# Autodesk Inventor assembly: Assembly5
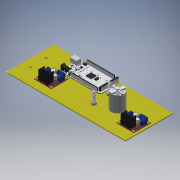
[picture p0: Inventor's stored thumbnail of the model, 180x180]
Saved by Autodesk Inventor 2019 (Build 230136000, 136)
## iProperties
Created: 2020-02-13
Part Number: Assembly5
Document SubType Name: Assembly
Designer: Dell
Author: Dell
## Documents named in this file (9)
- C:\Users\Dell\Documents\Assembly5.iam
- control.iam
- C:\Users\Dell\Documents\3dmodelling2.ipt
- C:\Users\Dell\Documents\bolt.ipt
- C:\Users\Dell\Documents\3dmodelling3.ipt
- C:\Users\Dell\Documents\nut2.ipt
- C:\Users\Dell\Documents\motordc2.ipt
- C:\Users\Dell\Documents\motordriver2.ipt
- C:\Users\Dell\Documents\arduinomega3.ipt
## Components (10 placed, 7 different names)
1. 3dmodelling2:1 — Rotational:1, Rotational:2, Rotational:3, Rotational:5, Mate:1, Mate:3
2. bolt:1 — Rotational:1
3. bolt:2 — Rotational:2, Rotational:4, Rotational:5, Rigid:1
4. 3dmodelling3:1 — Rotational:3, Rotational:4, Rotational:6, Rotational:7, Mate:2
5. nut2:1 — Rotational:6
6. nut2:2 — Rigid:1
7. motordc2:1 — Rotational:7
8. motordriver2:1 — Mate:2
9. motordriver2:2 — Mate:1
10. arduinomega3:1 — Mate:3
## Relationships (11: RevoluteJoint 7, Mate 3, WeldJoint 1)
- Rotational:1 [RevoluteJoint]: 3dmodelling2:1 ↔ bolt:1
- Rotational:2 [RevoluteJoint]: 3dmodelling2:1 ↔ bolt:2
- Rotational:3 [RevoluteJoint]: 3dmodelling2:1 ↔ 3dmodelling3:1
- Rotational:4 [RevoluteJoint]: bolt:2 ↔ 3dmodelling3:1
- Rotational:5 [RevoluteJoint]: 3dmodelling2:1 ↔ bolt:2
- Rigid:1 [WeldJoint]: bolt:2 ↔ nut2:2
- Rotational:6 [RevoluteJoint]: 3dmodelling3:1 ↔ nut2:1
- Rotational:7 [RevoluteJoint]: 3dmodelling3:1 ↔ motordc2:1
- Mate:1: 3dmodelling2:1 ↔ motordriver2:2
- Mate:2: 3dmodelling3:1 ↔ motordriver2:1
- Mate:3: 3dmodelling2:1 ↔ arduinomega3:1
